# Autodesk Inventor assembly: 092
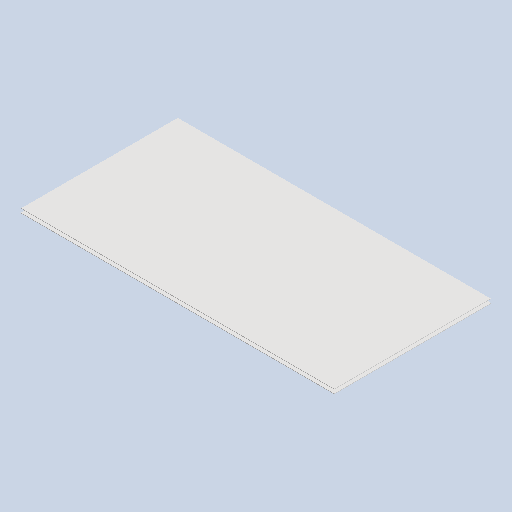
[picture p0: Inventor's stored thumbnail of the model, 512x512]
Saved by Autodesk Inventor 2026 (Build 300175000, 175)
## iProperties
Created: 2026-05-19
Part Number: 092
Document SubType Name: Assembly
Designer: user
Author: user
## Documents named in this file (4)
- C:\Users\user\Documents\Inventor\GBK-Gubkinskiy\Пол\092.iam
- C:\Users\user\Documents\Inventor\GBK-Gubkinskiy\Пол\0921.ipt
- C:\Users\user\Documents\Inventor\GBK-Gubkinskiy\Пол\0922.ipt
- C:\Users\user\Documents\Inventor\GBK-Gubkinskiy\Пол\0923.ipt
## Components (3 placed, 3 different names)
1. 0921:1 — Совмещение:1, Заподлицо:1, Заподлицо:2
2. 0922:1 — Жесткий:1, Совмещение:1, Заподлицо:1
3. 0923:1 — Жесткий:1, Заподлицо:2
## Relationships (4: Flush 2, WeldJoint 1, Mate 1)
- Жесткий:1 [WeldJoint]: 0922:1 ↔ 0923:1
- Совмещение:1 [Mate]: 0921:1 ↔ 0922:1
- Заподлицо:1 [Flush] (34 mm): 0921:1 ↔ 0922:1
- Заподлицо:2 [Flush] (34 mm): 0921:1 ↔ 0923:1
